# Autodesk Inventor assembly: MAX Motor Shaft Hubs
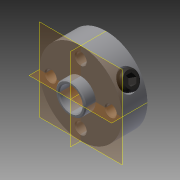
[picture p0: Inventor's stored thumbnail of the model, 180x180]
Saved by Autodesk Inventor 2015 (Build 190159000, 159)
## iProperties
Created: 2015-10-16
Part Number: MAX Motor Shaft Hubs
Document SubType Name: Assembly
Designer: Mason
Mass: 2.28336 g
Surface Area: 18.1886 cm^2
Volume: 2.28336 cm^3
Density: 1 g/cm^3
Author: Mason
## Documents named in this file (3)
- C:\Users\User\Documents\Inventor\Content Center Files\FTC\MAX Motor Shaft Hubs.iam
- C:\Users\User\Documents\Inventor\Content Center Files\FTC\ASM parts DO NOT TOUCH\MAX Motor Shaft Hubs Asm Parts\MAX Motor Shaft Hub Collar.ipt
- C:\Users\User\Documents\Inventor\Content Center Files\FTC\ASM parts DO NOT TOUCH\MAX Motor Shaft Hubs Asm Parts\MAX Motor Shaft Hub Screw.ipt
## Components (2 placed, 2 different names)
1. MAX Motor Shaft Hub Collar:1 — Mate:1
2. MAX Motor Shaft Hub Screw:1 — Mate:1
## Relationships (1: Mate 1)
- Mate:1: MAX Motor Shaft Hub Collar:1 ↔ MAX Motor Shaft Hub Screw:1
